# Autodesk Inventor assembly: IMUTrackerBase_8port_hub_asm
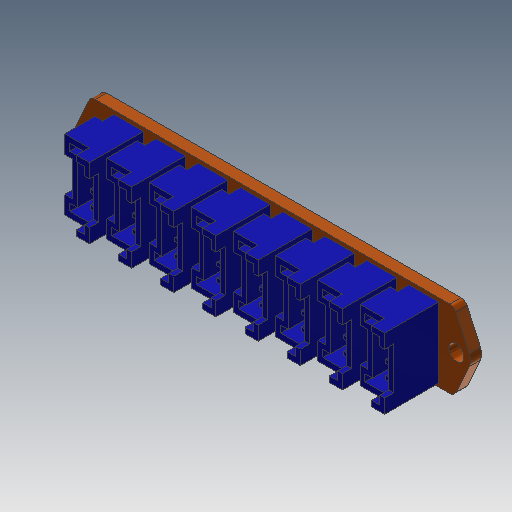
[picture p0: Inventor's stored thumbnail of the model, 512x512]
Saved by Autodesk Inventor 2019.4 (Build 234330000, 330)
## iProperties
Created: 2019-11-19
Part Number: IMUTrackerBase_8port_hub_asm
Material: 一般
Document SubType Name: Assembly
Designer: y6tada
Author: y6tada
## iProperties of the stored document B04B-PASK-1.ipt
Created: 2016-06-30
Part Number: B04B-PASK-1
Material: 一般
Description: STEP AP214
Document SubType Name: Modeling
Designer: y6tada
Density: 1 g/cm^3
Appearance: 既定
Sending System: SolidWorks 2009
Preprocessor: SwSTEP 2.0
Title: B04B-PASK-1(C³).STEP
Revision Number: ANY
## Documents named in this file (4)
- **C:\Workspace\QUIKS\Hardware\IMUTrackerBase\BASE_HUB_PCB\IMUTrackerBase_8port_hub_asm.iam*LocalDocs*xVwh4xy4eS2daungkB2ji3qwrKd*B04B-PASK-1.ipt
- C:\Workspace\QUIKS\Hardware\IMUTrackerBase\BASE_HUB_PCB\IMUTrackerBase_8port_hub_asm.iam
- C:\Workspace\QUIKS\Hardware\IMUTrackerBase\BASE_HUB_PCB\IMUTrackerBase_8port_hub_pcb.ipt
- C:\Workspace\QUIKS\Hardware\IMUTrackerBase\BASE_HUB_PCB\B04B-PASK-1.STEP
## Components (9 placed, 2 different names)
1. IMUTrackerBase_8port_hub_pcb:1 — メイト:1
2. B04B-PASK-1:1 — メイト:1, メイト:2, メイト:3
3. B04B-PASK-1:2
4. B04B-PASK-1:3
5. B04B-PASK-1:4
6. B04B-PASK-1:5
7. B04B-PASK-1:6
8. B04B-PASK-1:7
9. B04B-PASK-1:8
## Component patterns: (8 elements, first: B04B-PASK-1:1)
## Relationships (3: Mate 3)
- メイト:1 [Mate]: IMUTrackerBase_8port_hub_pcb:1 ↔ B04B-PASK-1:1
- メイト:2 [Mate] (-20.55 mm): B04B-PASK-1:1
- メイト:3 [Mate]: B04B-PASK-1:1
